# Autodesk Inventor assembly: sostenedor
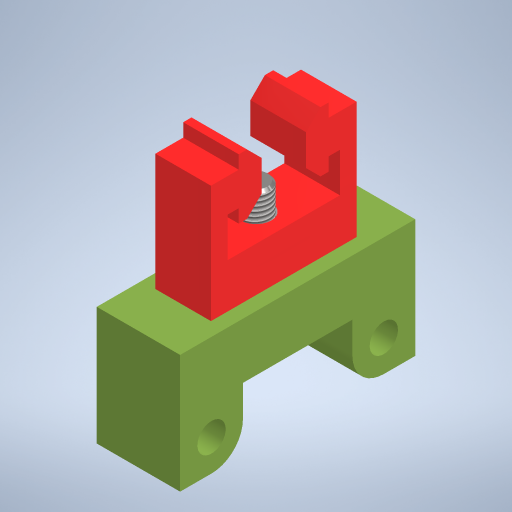
[picture p0: Inventor's stored thumbnail of the model, 512x512]
Saved by Autodesk Inventor 2023.2 (Build 272271030, 271C)
## iProperties
Created: 2023-03-04
Part Number: sostenedor
Document SubType Name: Assembly
Designer: Cris Pat
Author: Cris Pat
## Documents named in this file (4)
- C:\Users\Cris Pat\Desktop\U\Semestre 9\disenio e innovacion\CAD\Hbot\sostenedor.iam
- C:\Users\Cris Pat\Desktop\U\Semestre 9\disenio e innovacion\CAD\Hbot\sostenedor_part1.ipt
- C:\Users\Cris Pat\Desktop\U\Semestre 9\disenio e innovacion\CAD\Hbot\sostenedor_part2.ipt
- C:\Users\Cris Pat\Desktop\U\Semestre 9\disenio e innovacion\CAD\Hbot\libreria\en-US\DIN 84\DIN 84 - M5 x 20.ipt
## Components (3 placed, 3 different names)
1. sostenedor_part1:1 — Rigid:1
2. sostenedor_part2:1 — Rigid:1, Insert:1
3. DIN 84 - replaced by DIN EN ISO 1207 M5 x 20:1 — Insert:1
## Relationships (2: WeldJoint 1, Insert 1)
- Rigid:1 [WeldJoint]: sostenedor_part1:1 ↔ sostenedor_part2:1
- Insert:1: sostenedor_part2:1 ↔ DIN 84 - replaced by DIN EN ISO 1207 M5 x 20:1
